# Autodesk Inventor assembly: Claw Plate Assy
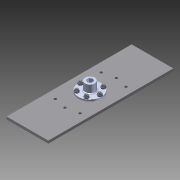
[picture p0: Inventor's stored thumbnail of the model, 180x180]
Saved by Autodesk Inventor 2014 (Build 180170000, 170)
## iProperties
Created: 2015-01-25
Part Number: Claw Plate Assy
Document SubType Name: Assembly
Designer: chappelled
Author: chappelled
## Documents named in this file (5)
- C:\Users\chappelled\Documents\Inventor\Claw\Claw Plate Assy.iam
- C:\Users\chappelled\Documents\Inventor\Claw\Claw Plate.ipt
- C:\Users\chappelled\Documents\Inventor\Claw\Imported Components\am-0096a+500+Hex+Hub+r2\am-0096a+500+Hex+Hub+r2.ipt
- C:\Users\chappelled\Documents\Inventor\Claw\Claw Plate Assy\Design Accelerator\Bolted Connection1.iam
- C:\Users\chappelled\Documents\Inventor\Claw\Imported Components\1494A420 Hinge\1494A420 Hinge.ipt
## Components (5 placed, 4 different names)
1. Claw Plate:1 — Mate:1, Mate:2, Mate:3, Mate:4, Mate:5, Mate:6, Flush:1, Mate:7, Mate:8, Mate:9
2. am-0096a+500+Hex+Hub+r2:1 — Mate:1, Mate:2, Mate:3
3. Bolted Connection:1 [sub-assembly] — Mate:4, Mate:5
4. 1494A420 Hinge:1 — Mate:6
5. 1494A420 Hinge:2 — Mate:7, Mate:8, Mate:9
## Relationships (10: Mate 9, Flush 1)
- Mate:1: Claw Plate:1 ↔ am-0096a+500+Hex+Hub+r2:1
- Mate:2: Claw Plate:1 ↔ am-0096a+500+Hex+Hub+r2:1
- Mate:3: Claw Plate:1 ↔ am-0096a+500+Hex+Hub+r2:1
- Mate:4: Claw Plate:1 ↔ Bolted Connection:1
- Mate:5: Claw Plate:1 ↔ Bolted Connection:1
- Mate:6: Claw Plate:1 ↔ 1494A420 Hinge:1
- Flush:1 (-152.4 mm): Claw Plate:1
- Mate:7: Claw Plate:1 ↔ 1494A420 Hinge:2
- Mate:8: Claw Plate:1 ↔ 1494A420 Hinge:2
- Mate:9: Claw Plate:1 ↔ 1494A420 Hinge:2
